# Autodesk Inventor assembly: Sestava1
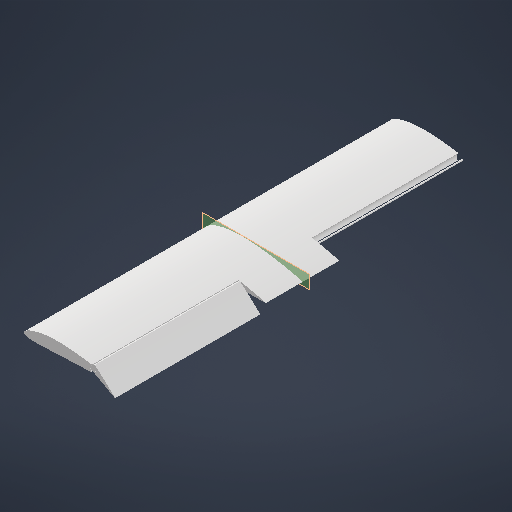
[picture p0: Inventor's stored thumbnail of the model, 512x512]
Saved by Autodesk Inventor 2026 (Build 300175050, 175E)
## iProperties
Created: 2026-01-17
Part Number: Sestava1
Document SubType Name: Assembly
Designer: marti
Author: marti
## Documents named in this file (4)
- F:\Ročníkovka\RP_Svitek\3d model\Sestava1.iam
- F:\Ročníkovka\RP_Svitek\3d model\pokus 1 .ipt
- F:\Ročníkovka\RP_Svitek\3d model\tyč.ipt
- F:\Ročníkovka\RP_Svitek\3d model\pokus 1 flap 4412 .ipt
## Components (3 placed, 3 different names)
1. pokus 1 :1 — Stejný směr:1, Vložit:1
2. tyč:1 — Vložit:1, Rotační:1
3. pokus 1 flap 4412 :1 — Rotační:1
## Relationships (3: Flush 1, Insert 1, RevoluteJoint 1)
- Stejný směr:1 [Flush]: pokus 1 :1
- Vložit:1 [Insert] (-300 mm): pokus 1 :1 ↔ tyč:1
- Rotační:1 [RevoluteJoint]: tyč:1 ↔ pokus 1 flap 4412 :1
